# Autodesk Inventor assembly: Final Assembly
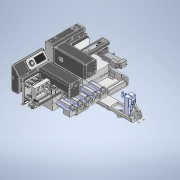
[picture p0: Inventor's stored thumbnail of the model, 180x180]
Saved by Autodesk Inventor 2022 (Build 260153000, 153)
## iProperties
Created: 2021-11-30
Part Number: Final Assembly
Document SubType Name: Assembly
Designer: efred
Author: efred
## Documents named in this file (59)
- C:\Users\efred\OneDrive - Imperial College London\Old Shit\ROBOICP\Final Assembly\Final Assembly.iam
- C:\Users\efred\OneDrive - Imperial College London\Old Shit\ROBOICP\Final Assembly\Linear Rail Base.ipt
- C:\Users\efred\OneDrive - Imperial College London\Old Shit\ROBOICP\Final Assembly\Linear Rail Carriage.ipt
- C:\Users\efred\OneDrive - Imperial College London\Old Shit\ROBOICP\Final Assembly\Linear Rail motor.ipt
- C:\Users\efred\OneDrive - Imperial College London\Old Shit\ROBOICP\Final Assembly\Linear Rail End Cap.ipt
- C:\Users\efred\OneDrive - Imperial College London\Old Shit\ROBOICP\Final Assembly\Linear Rail Front Plate.ipt
- C:\Users\efred\OneDrive - Imperial College London\Old Shit\ROBOICP\Final Assembly\endcap insert.ipt
- C:\Users\efred\OneDrive - Imperial College London\Old Shit\ROBOICP\Final Assembly\endcap insert_MIR.ipt
- C:\Users\efred\OneDrive - Imperial College London\Old Shit\ROBOICP\Final Assembly\backboard.ipt
- C:\Users\efred\OneDrive - Imperial College London\Old Shit\ROBOICP\Final Assembly\backboard_MIR.ipt
- C:\Users\efred\OneDrive - Imperial College London\Old Shit\ROBOICP\Final Assembly\Syringe adapter to rail.ipt
- C:\Users\efred\OneDrive - Imperial College London\Old Shit\ROBOICP\Final Assembly\SyringeHolder.ipt
- C:\Users\efred\OneDrive - Imperial College London\Old Shit\ROBOICP\Final Assembly\Guide rod bottom stand (independent).ipt
- C:\Users\efred\OneDrive - Imperial College London\Old Shit\ROBOICP\Final Assembly\Linear Rail Frame Bracket.ipt
- C:\Users\efred\OneDrive - Imperial College London\Old Shit\ROBOICP\Final Assembly\Linear Rail Frame Bracket_MIR.ipt
- C:\Users\efred\OneDrive - Imperial College London\Old Shit\ROBOICP\Final Assembly\Lower Support.ipt
- C:\Users\efred\OneDrive - Imperial College London\Old Shit\ROBOICP\Final Assembly\Lower Support_MIR.ipt
- C:\Users\efred\OneDrive - Imperial College London\Old Shit\ROBOICP\Final Assembly\Linear actuator piston.ipt
- C:\Users\efred\OneDrive - Imperial College London\Old Shit\ROBOICP\Final Assembly\linear actuator conrod.ipt
- C:\Users\efred\OneDrive - Imperial College London\Old Shit\ROBOICP\Final Assembly\6x250 steel rod.ipt
- C:\Users\efred\OneDrive - Imperial College London\Old Shit\ROBOICP\Final Assembly\cantilever.ipt
- C:\Users\efred\OneDrive - Imperial College London\Old Shit\ROBOICP\Final Assembly\Servo head assembly.iam
- C:\Users\efred\OneDrive - Imperial College London\Old Shit\ROBOICP\Final Assembly\Conrod.ipt
- C:\Users\efred\OneDrive - Imperial College London\Old Shit\ROBOICP\Final Assembly\Syringe Lower.ipt
- C:\Users\efred\OneDrive - Imperial College London\Old Shit\ROBOICP\Final Assembly\Plunger Assembly.iam
- C:\Users\efred\OneDrive - Imperial College London\Old Shit\ROBOICP\Final Assembly\Dilution Printer.iam
- C:\Users\efred\OneDrive - Imperial College London\Old Shit\ROBOICP\Final Assembly\Bed plate.ipt
- C:\Users\efred\OneDrive - Imperial College London\Old Shit\ROBOICP\Final Assembly\Nema17(SY42STH47-1684A)singelshaft.ipt
- C:\Users\efred\OneDrive - Imperial College London\Old Shit\ROBOICP\Final Assembly\Rotating Vial Holder EXP Slice.ipt
- C:\Users\efred\OneDrive - Imperial College London\Old Shit\ROBOICP\Final Assembly\small Vial.ipt
- C:\Users\efred\OneDrive - Imperial College London\Old Shit\ROBOICP\Final Assembly\L298N.ipt
- C:\Users\efred\OneDrive - Imperial College London\Old Shit\ROBOICP\Final Assembly\Reaction Printer.iam
- C:\Users\efred\OneDrive - Imperial College London\Old Shit\ROBOICP\Final Assembly\Raspberry Pi 3.ipt
- C:\Users\efred\OneDrive - Imperial College London\Old Shit\ROBOICP\Final Assembly\linear actuator.ipt
- C:\Users\efred\OneDrive - Imperial College London\Old Shit\ROBOICP\Final Assembly\Power brick assembly.iam
- C:\Users\efred\OneDrive - Imperial College London\Old Shit\ROBOICP\Final Assembly\printer power brick assembly.iam
- C:\Users\efred\OneDrive - Imperial College London\Old Shit\ROBOICP\Final Assembly\dilution system bracket.ipt
- C:\Users\efred\OneDrive - Imperial College London\Old Shit\ROBOICP\Final Assembly\dilution system bracket_MIR.ipt
- C:\Users\efred\OneDrive - Imperial College London\Old Shit\ROBOICP\Final Assembly\pivot module base.ipt
- C:\Users\efred\OneDrive - Imperial College London\Old Shit\ROBOICP\Final Assembly\pivot module stalk.ipt
- C:\Users\efred\OneDrive - Imperial College London\Old Shit\ROBOICP\Final Assembly\TB6600 - Driver Motor de Passo 4A.ipt
- C:\Users\efred\OneDrive - Imperial College London\Old Shit\ROBOICP\Final Assembly\persitaltic pump assembly.iam
- C:\Users\efred\OneDrive - Imperial College London\Old Shit\ROBOICP\Final Assembly\ArduinoMega_STEP_AP203.ipt
- C:\Users\efred\OneDrive - Imperial College London\Old Shit\ROBOICP\Final Assembly\electronics box.ipt
- C:\Users\efred\Downloads\Breadboard.ipt
- C:\Users\efred\OneDrive - Imperial College London\Old Shit\ROBOICP\Final Assembly\sump.ipt
- C:\Users\efred\Downloads\beaker holder.ipt
- C:\Users\efred\OneDrive - Imperial College London\Old Shit\ROBOICP\Final Assembly\Keyes KY 019 Montaj.ipt
- C:\Users\efred\OneDrive - Imperial College London\Old Shit\ROBOICP\Final Assembly\Micropippete mount assembly.iam
- C:\Users\efred\OneDrive - Imperial College London\Old Shit\ROBOICP\Final Assembly\Solids Feeder Head Assembly.iam
- C:\Users\efred\OneDrive - Imperial College London\Old Shit\ROBOICP\Final Assembly\male head_1.75R.ipt
- C:\Users\efred\OneDrive - Imperial College London\Old Shit\ROBOICP\Final Assembly\new top 4.0.ipt
- C:\Users\efred\OneDrive - Imperial College London\Old Shit\ROBOICP\Final Assembly\vial.ipt
- C:\Users\efred\OneDrive - Imperial College London\Old Shit\ROBOICP\Final Assembly\female mixing head.ipt
- C:\Users\efred\OneDrive - Imperial College London\Old Shit\ROBOICP\Final Assembly\Mixer.ipt
- C:\Users\efred\OneDrive - Imperial College London\Old Shit\ROBOICP\Final Assembly\vial holder 2.ipt
- C:\Users\efred\OneDrive - Imperial College London\Old Shit\ROBOICP\Final Assembly\hopper motor holder.ipt
- C:\Users\efred\OneDrive - Imperial College London\Old Shit\ROBOICP\Final Assembly\motor.ipt
- C:\Users\efred\OneDrive - Imperial College London\Old Shit\ROBOICP\Final Assembly\motor viber.ipt
## Components (80 placed, 58 different names)
1. Linear Rail Base:1 — Flush:1, Mate:1, Mate:2, Flush:2, Mate:3, Mate:4, Mate:5, Mate:6, Flush:6, Mate:18, Flush:13, Flush:70, Flush:71
2. Linear Rail Carriage:1 — Mate:5, Mate:6, Mate:14, Angle:2, Flush:9, Flush:10, Flush:12
3. Linear Rail motor:1 — Mate:7, Angle:1, Mate:8
4. Linear Rail End Cap:1 — Flush:2, Mate:3, Mate:4, Flush:3, Mate:126
5. Linear Rail Front Plate:1 — Flush:1, Mate:1, Mate:2, Mate:7, Angle:1, Mate:8, Mate:17, Mate:71, Mate:72, Flush:72, Mate:125
6. endcap insert:1 — Flush:4, Flush:5, Flush:15
7. endcap insert_MIR:1 — Mate:9, Mate:10, Mate:71, Mate:72, Flush:72, Mate:73, Mate:75
8. backboard:1 — Flush:7, Flush:71, Mate:73, Mate:74, Mate:79, Mate:80, Mate:81
9. backboard_MIR:1 — Mate:11, Flush:14, Flush:70, Mate:76, Mate:77, Mate:78, Mate:147, Flush:130
10. Syringe adapter to rail:1 — Mate:14, Angle:2, Flush:9, Flush:10, Mate:15, Mate:16, Mate:17, Mate:125, Mate:126
11. SyringeHolder:1 — Mate:15, Flush:12, Mate:16, Mate:45, Mate:46, Angle:3
12. Guide rod bottom stand (independent):1 — Mate:18, Flush:13, Mate:30, Mate:32, Mate:37, Mate:41, Mate:42, Mate:49, Flush:68, Mate:68, Mate:69, Mate:70, Mate:91, Flush:75, Mate:101, Flush:103, Mate:102, Flush:104
13. Linear Rail Frame Bracket:1 — Flush:15
14. Linear Rail Frame Bracket_MIR:1 — Mate:74, Mate:75
15. Lower Support:1 — Flush:16, Flush:17, Mate:79, Mate:80, Mate:81, Flush:81, Mate:160
16. Lower Support_MIR:1 — Flush:17, Flush:69, Mate:76, Mate:77, Mate:78, Angle:5, Mate:92, Flush:83, Flush:105, Mate:104, Mate:105, Mate:148, Flush:133, Flush:164
17. Linear actuator piston:1 — Mate:67, Mate:103
18. 6x250 steel rod:1 — Mate:30, Mate:43, Mate:70
19. cantilever:1 — Mate:32, Mate:39, Mate:66, Mate:69
20. Servo head assembly:1 [sub-assembly] — Mate:38, Mate:43, Mate:68, Mate:89, Mate:91
21. Conrod:1 — Mate:37, Mate:38, Mate:39
22. 6x250 steel rod:2 — Mate:41, Mate:42
23. Dilution Printer:1 [sub-assembly] — Flush:69, Mate:82, Mate:83, Mate:84, Angle:4, Angle:5, Mate:92, Flush:83, Flush:113, Mate:166, Mate:167, Mate:168
24. Bed plate:1 — Mate:55, Mate:56, Mate:57, Mate:82, Mate:83, Mate:84, Mate:86, Mate:144, Mate:145
25. Nema17(SY42STH47-1684A)singelshaft:1 — Mate:55, Mate:56, Mate:57, Mate:85
26. linear actuator conrod:1 — Flush:68, Mate:66, Mate:67
27. Rotating Vial Holder EXP Slice:1 — Mate:85, Mate:86, Angle:4, Mate:87, Mate:88
28. small Vial:1 — Mate:87, Mate:88, Mate:89
29. Reaction Printer:1 [sub-assembly] — Flush:81, Mate:159, Mate:160, Mate:171, Mate:172, Flush:177, Flush:178, Flush:180, Mate:173, Mate:174, Flush:181, Flush:182, Mate:177, Flush:184, Flush:188
30. Raspberry Pi 3:1 — Flush:158, Flush:159, Mate:158
31. linear actuator:1 — Mate:101, Flush:103, Mate:102, Flush:104, Mate:103
32. Power brick assembly:1 [sub-assembly] — Mate:106, Flush:106, Flush:107
33. dilution system bracket:1 — Flush:114, Flush:115, Flush:168, Mate:159
34. dilution system bracket_MIR:1 — Mate:123, Mate:124, Flush:167, Flush:173
35. pivot module base:1 — Flush:116, Flush:117
36. pivot module stalk:1 — Flush:118, Flush:119
37. small Vial:2 — Mate:144, Mate:145
38. persitaltic pump assembly:1 [sub-assembly] — Mate:147, Flush:130, Mate:148
39. ArduinoMega_STEP_AP203:1 — Mate:155, Mate:156, Mate:157
40. electronics box:1 — Mate:152, Flush:136, Flush:137, Mate:153, Mate:154, Mate:162, Tangent:5, Flush:156, Mate:161, Mate:156, Flush:159, Mate:158, Mate:163, Mate:164, Mate:165
41. Breadboard:2 — Mate:153, Flush:156, Mate:161, Flush:158, Mate:157
42. sump:1 — Flush:165, Flush:166, Flush:167, Flush:168
43. beaker holder:1 — Flush:174
44. Keyes KY 019 Montaj:1 — Mate:163, Mate:164, Mate:165
45. Micropippete mount assembly:1 [sub-assembly] — Mate:166, Mate:167, Mate:168
46. Solids Feeder Head Assembly:1 [sub-assembly] — Mate:171, Mate:172, Flush:177, Flush:179, Flush:180, Flush:189, Mate:188, Mate:189
47. male head_1.75R:1 — Mate:173, Mate:174, Flush:183, Mate:178
48. new top 4.0:1 — Flush:181, Flush:182, Mate:175, Mate:178, Flush:187, Mate:182, Mate:183, Flush:192, Mate:192
49. female mixing head:1 — Flush:187, Angle:6, Mate:190, Mate:191
50. Mixer:1 — Angle:6, Mate:190, Mate:191
51. vial holder 2:1 — Flush:188
52. hopper motor holder:1 — Flush:190, Flush:191, Mate:188, Mate:189, Mate:194, Flush:197
53. hopper motor holder:2 — Mate:182, Mate:183, Flush:192, Mate:185, Flush:194
54. motor:2 — Mate:185, Flush:194, Mate:186, Flush:195
55. motor viber:1 — Mate:186, Flush:195
56. motor:3 — Mate:194, Flush:197
57. motor viber:2
58. Syringe Lower:1 — Mate:45, Mate:46, Angle:3, Mate:47, Mate:48
59. Syringe Lower:2
60. Syringe Lower:3
61. Syringe Lower:4
62. Syringe Lower:5
63. Plunger Assembly:1 [sub-assembly] — Mate:47, Mate:48, Mate:49
64. Plunger Assembly:2 [sub-assembly]
65. Plunger Assembly:3 [sub-assembly]
66. Plunger Assembly:4 [sub-assembly]
67. Plunger Assembly:5 [sub-assembly]
68. printer power brick assembly:1 [sub-assembly] — Flush:105, Mate:104, Mate:105
69. printer power brick assembly:2 [sub-assembly] — Mate:106, Flush:106, Flush:107
70. L298N:1 — Mate:152, Flush:136, Flush:137
71. L298N:2
72. L298N:3 — Mate:155
73. TB6600 - Driver Motor de Passo 4A:1 — Mate:154, Mate:162, Tangent:5
74. TB6600 - Driver Motor de Passo 4A:2
75. vial:1 — Mate:175, Mate:177, Mate:192
76. vial:2
77. vial:3
78. vial:4
79. vial:5
80. vial:6
## Component patterns: (5 elements, first: Syringe Lower:1), (5 elements, first: Plunger Assembly:1), (2 elements, first: printer power brick assembly:1), (3 elements, first: L298N:1), (2 elements, first: TB6600 - Driver Motor de Passo 4A:1), (6 elements, first: vial:1)
## Relationships (181: Mate 107, Flush 67, Angle 6, Tangent 1)
- Flush:1: Linear Rail Base:1 ↔ Linear Rail Front Plate:1
- Mate:1 (3.2 mm): Linear Rail Base:1 ↔ Linear Rail Front Plate:1
- Mate:2: Linear Rail Base:1 ↔ Linear Rail Front Plate:1
- Flush:2: Linear Rail Base:1 ↔ Linear Rail End Cap:1
- Mate:3 (3.2 mm): Linear Rail Base:1 ↔ Linear Rail End Cap:1
- Mate:4: Linear Rail Base:1 ↔ Linear Rail End Cap:1
- Mate:5 (1 mm): Linear Rail Base:1 ↔ Linear Rail Carriage:1
- Mate:6: Linear Rail Base:1 ↔ Linear Rail Carriage:1
- Mate:7: Linear Rail motor:1 ↔ Linear Rail Front Plate:1
- Angle:1 (0 deg): Linear Rail motor:1 ↔ Linear Rail Front Plate:1
- Mate:8: Linear Rail motor:1 ↔ Linear Rail Front Plate:1
- Flush:3 (0.1 mm): Linear Rail End Cap:1
- Flush:4: endcap insert:1
- Flush:5: endcap insert:1
- Mate:9: endcap insert_MIR:1
- Mate:10: endcap insert_MIR:1
- Flush:6 (0.1 mm): Linear Rail Base:1
- Flush:7 (0.1 mm): backboard:1
- Mate:11 (0.1 mm): backboard_MIR:1
- Mate:14 (0.1 mm): Linear Rail Carriage:1 ↔ Syringe adapter to rail:1
- Angle:2 (0 deg): Linear Rail Carriage:1 ↔ Syringe adapter to rail:1
- Flush:9: Linear Rail Carriage:1 ↔ Syringe adapter to rail:1
- Flush:10: Linear Rail Carriage:1 ↔ Syringe adapter to rail:1
- Mate:15 (0.1 mm): Syringe adapter to rail:1 ↔ SyringeHolder:1
- Flush:12: Linear Rail Carriage:1 ↔ SyringeHolder:1
- Mate:16 (0.1 mm): Syringe adapter to rail:1 ↔ SyringeHolder:1
- Mate:17 (1 mm): Linear Rail Front Plate:1 ↔ Syringe adapter to rail:1
- Mate:18 (0.1 mm): Linear Rail Base:1 ↔ Guide rod bottom stand (independent):1
- Flush:13 (-252.9 mm): Linear Rail Base:1 ↔ Guide rod bottom stand (independent):1
- Flush:14 (0.1 mm): backboard_MIR:1
- Flush:15: endcap insert:1 ↔ Linear Rail Frame Bracket:1
- Flush:16: Lower Support:1
- Flush:17: Lower Support:1 ↔ Lower Support_MIR:1
- Mate:30 (0.1 mm): Guide rod bottom stand (independent):1 ↔ 6x250 steel rod:1
- Mate:32: Guide rod bottom stand (independent):1 ↔ cantilever:1
- Mate:37: Guide rod bottom stand (independent):1 ↔ Conrod:1
- Mate:38: Servo head assembly:1 ↔ Conrod:1
- Mate:39: cantilever:1 ↔ Conrod:1
- Mate:41 (0.1 mm): Guide rod bottom stand (independent):1 ↔ 6x250 steel rod:2
- Mate:42: Guide rod bottom stand (independent):1 ↔ 6x250 steel rod:2
- Mate:43: 6x250 steel rod:1 ↔ Servo head assembly:1
- Mate:45 (0.1 mm): SyringeHolder:1 ↔ Syringe Lower:1
- Mate:46: SyringeHolder:1 ↔ Syringe Lower:1
- Angle:3 (0 deg): SyringeHolder:1 ↔ Syringe Lower:1
- Mate:47: Syringe Lower:1 ↔ Plunger Assembly:1
- Mate:48 (9.6 mm): Syringe Lower:1 ↔ Plunger Assembly:1
- Mate:49: Guide rod bottom stand (independent):1 ↔ Plunger Assembly:1
- Mate:55 (0.1 mm): Bed plate:1 ↔ Nema17(SY42STH47-1684A)singelshaft:1
- Mate:56 (0.1 mm): Bed plate:1 ↔ Nema17(SY42STH47-1684A)singelshaft:1
- Mate:57 (0.1 mm): Bed plate:1 ↔ Nema17(SY42STH47-1684A)singelshaft:1
- Flush:68: Guide rod bottom stand (independent):1 ↔ linear actuator conrod:1
- Mate:66: cantilever:1 ↔ linear actuator conrod:1
- Mate:67: Linear actuator piston:1 ↔ linear actuator conrod:1
- Mate:68: Guide rod bottom stand (independent):1 ↔ Servo head assembly:1
- Mate:69: Guide rod bottom stand (independent):1 ↔ cantilever:1
- Mate:70: Guide rod bottom stand (independent):1 ↔ 6x250 steel rod:1
- Flush:69: Lower Support_MIR:1 ↔ Dilution Printer:1
- Flush:70: Linear Rail Base:1 ↔ backboard_MIR:1
- Flush:71: Linear Rail Base:1 ↔ backboard:1
- Mate:71 (0.1 mm): Linear Rail Front Plate:1 ↔ endcap insert_MIR:1
- Mate:72: Linear Rail Front Plate:1 ↔ endcap insert_MIR:1
- Flush:72: Linear Rail Front Plate:1 ↔ endcap insert_MIR:1
- Mate:73: endcap insert_MIR:1 ↔ backboard:1
- Mate:74: backboard:1 ↔ Linear Rail Frame Bracket_MIR:1
- Mate:75: endcap insert_MIR:1 ↔ Linear Rail Frame Bracket_MIR:1
- Mate:76 (0.1 mm): backboard_MIR:1 ↔ Lower Support_MIR:1
- Mate:77 (0.1 mm): backboard_MIR:1 ↔ Lower Support_MIR:1
- Mate:78 (0.1 mm): backboard_MIR:1 ↔ Lower Support_MIR:1
- Mate:79 (0.1 mm): backboard:1 ↔ Lower Support:1
- Mate:80 (0.1 mm): backboard:1 ↔ Lower Support:1
- Mate:81 (0.1 mm): backboard:1 ↔ Lower Support:1
- Mate:82 (0.1 mm): Dilution Printer:1 ↔ Bed plate:1
- Mate:83: Dilution Printer:1 ↔ Bed plate:1
- Mate:84: Dilution Printer:1 ↔ Bed plate:1
- Mate:85: Nema17(SY42STH47-1684A)singelshaft:1 ↔ Rotating Vial Holder EXP Slice:1
- Mate:86 (10 mm): Bed plate:1 ↔ Rotating Vial Holder EXP Slice:1
- Angle:4 (20 deg): Dilution Printer:1 ↔ Rotating Vial Holder EXP Slice:1
- Mate:87: Rotating Vial Holder EXP Slice:1 ↔ small Vial:1
- Mate:88 (0.1 mm): Rotating Vial Holder EXP Slice:1 ↔ small Vial:1
- Mate:89: Servo head assembly:1 ↔ small Vial:1
- Angle:5 (0 deg): Lower Support_MIR:1 ↔ Dilution Printer:1
- Mate:91: Guide rod bottom stand (independent):1 ↔ Servo head assembly:1
- Mate:92 (58 mm): Lower Support_MIR:1 ↔ Dilution Printer:1
- Flush:75 (0.1 mm): Guide rod bottom stand (independent):1
- Flush:81: Lower Support:1 ↔ Reaction Printer:1
- Flush:83 (108 mm): Lower Support_MIR:1 ↔ Dilution Printer:1
- Mate:101 (0.1 mm): Guide rod bottom stand (independent):1 ↔ linear actuator:1
- Flush:103: Guide rod bottom stand (independent):1 ↔ linear actuator:1
- Mate:102 (-50 mm): Guide rod bottom stand (independent):1 ↔ linear actuator:1
- Flush:104: Guide rod bottom stand (independent):1 ↔ linear actuator:1
- Mate:103: Linear actuator piston:1 ↔ linear actuator:1
- Flush:105: Lower Support_MIR:1 ↔ printer power brick assembly:1
- Mate:104 (0.1 mm): Lower Support_MIR:1 ↔ printer power brick assembly:1
- Mate:105 (0.1 mm): Lower Support_MIR:1 ↔ printer power brick assembly:1
- Mate:106 (1 mm): Power brick assembly:1 ↔ printer power brick assembly:2
- Flush:106: Power brick assembly:1 ↔ printer power brick assembly:2
- Flush:107: Power brick assembly:1 ↔ printer power brick assembly:2
- Flush:113 (0.1 mm): Dilution Printer:1
- Flush:114: dilution system bracket:1
- Flush:115: dilution system bracket:1
- Mate:123: dilution system bracket_MIR:1
- Mate:124: dilution system bracket_MIR:1
- Flush:116: pivot module base:1
- Flush:117 (0.1 mm): pivot module base:1
- Flush:118: pivot module stalk:1
- Flush:119: pivot module stalk:1
- Mate:125: Linear Rail Front Plate:1 ↔ Syringe adapter to rail:1
- Mate:126: Linear Rail End Cap:1 ↔ Syringe adapter to rail:1
- Mate:144: Bed plate:1 ↔ small Vial:2
- Mate:145 (0.1 mm): Bed plate:1 ↔ small Vial:2
- Mate:147 (0.1 mm): backboard_MIR:1 ↔ persitaltic pump assembly:1
- Flush:130 (15 mm): backboard_MIR:1 ↔ persitaltic pump assembly:1
- Mate:148 (0.1 mm): Lower Support_MIR:1 ↔ persitaltic pump assembly:1
- Flush:133 (0.1 mm): Lower Support_MIR:1
- Mate:152 (5 mm): electronics box:1 ↔ L298N:1
- Flush:136 (1 mm): electronics box:1 ↔ L298N:1
- Flush:137 (10 mm): electronics box:1 ↔ L298N:1
- Mate:153 (0.1 mm): electronics box:1 ↔ Breadboard:2
- Mate:154 (0.1 mm): electronics box:1 ↔ TB6600 - Driver Motor de Passo 4A:1
- Mate:162 (10 mm): electronics box:1 ↔ TB6600 - Driver Motor de Passo 4A:1
- Tangent:5: electronics box:1 ↔ TB6600 - Driver Motor de Passo 4A:1
- Flush:156 (1 mm): electronics box:1 ↔ Breadboard:2
- Mate:161 (1 mm): electronics box:1 ↔ Breadboard:2
- Mate:155 (5 mm): ArduinoMega_STEP_AP203:1 ↔ L298N:3
- Mate:156 (5 mm): ArduinoMega_STEP_AP203:1 ↔ electronics box:1
- Flush:158 (30 mm): Raspberry Pi 3:1 ↔ Breadboard:2
- Flush:159: Raspberry Pi 3:1 ↔ electronics box:1
- Mate:157 (1 mm): ArduinoMega_STEP_AP203:1 ↔ Breadboard:2
- Mate:158 (5 mm): Raspberry Pi 3:1 ↔ electronics box:1
- Flush:164 (0.1 mm): Lower Support_MIR:1
- Flush:165: sump:1
- Flush:166: sump:1
- Flush:167 (0.1 mm): dilution system bracket_MIR:1 ↔ sump:1
- Flush:168 (0.1 mm): dilution system bracket:1 ↔ sump:1
- Flush:173 (0.1 mm): dilution system bracket_MIR:1
- Flush:174: beaker holder:1
- Mate:159 (25 mm): Reaction Printer:1 ↔ dilution system bracket:1
- Mate:160 (30 mm): Lower Support:1 ↔ Reaction Printer:1
- Mate:163: electronics box:1 ↔ Keyes KY 019 Montaj:1
- Mate:164: electronics box:1 ↔ Keyes KY 019 Montaj:1
- Mate:165 (1 mm): electronics box:1 ↔ Keyes KY 019 Montaj:1
- Mate:166 (0.1 mm): Dilution Printer:1 ↔ Micropippete mount assembly:1
- Mate:167: Dilution Printer:1 ↔ Micropippete mount assembly:1
- Mate:168: Dilution Printer:1 ↔ Micropippete mount assembly:1
- Mate:171 (5 mm): Reaction Printer:1 ↔ Solids Feeder Head Assembly:1
- Mate:172 (0.1 mm): Reaction Printer:1 ↔ Solids Feeder Head Assembly:1
- Flush:177: Reaction Printer:1 ↔ Solids Feeder Head Assembly:1
- Flush:178 (0.1 mm): Reaction Printer:1
- Flush:179: Solids Feeder Head Assembly:1
- Flush:180 (0.1 mm): Reaction Printer:1 ↔ Solids Feeder Head Assembly:1
- Mate:173: Reaction Printer:1 ↔ male head_1.75R:1
- Mate:174 (0.1 mm): Reaction Printer:1 ↔ male head_1.75R:1
- Flush:181: Reaction Printer:1 ↔ new top 4.0:1
- Flush:182 (4 mm): Reaction Printer:1 ↔ new top 4.0:1
- Mate:175: new top 4.0:1 ↔ vial:1
- Mate:177 (0.1 mm): Reaction Printer:1 ↔ vial:1
- Flush:183: male head_1.75R:1
- Flush:184 (0.1 mm): Reaction Printer:1
- Mate:178 (1 mm): male head_1.75R:1 ↔ new top 4.0:1
- Flush:187: new top 4.0:1 ↔ female mixing head:1
- Flush:188: Reaction Printer:1 ↔ vial holder 2:1
- Flush:189 (0.1 mm): Solids Feeder Head Assembly:1
- Flush:190: hopper motor holder:1
- Flush:191: hopper motor holder:1
- Mate:182 (0.1 mm): new top 4.0:1 ↔ hopper motor holder:2
- Mate:183 (0.1 mm): new top 4.0:1 ↔ hopper motor holder:2
- Flush:192: new top 4.0:1 ↔ hopper motor holder:2
- Mate:185: hopper motor holder:2 ↔ motor:2
- Flush:194: hopper motor holder:2 ↔ motor:2
- Mate:186: motor:2 ↔ motor viber:1
- Flush:195: motor:2 ↔ motor viber:1
- Mate:188 (0.1 mm): Solids Feeder Head Assembly:1 ↔ hopper motor holder:1
- Mate:189: Solids Feeder Head Assembly:1 ↔ hopper motor holder:1
- Angle:6 (0 deg): female mixing head:1 ↔ Mixer:1
- Mate:190 (0.1 mm): female mixing head:1 ↔ Mixer:1
- Mate:191: female mixing head:1 ↔ Mixer:1
- Mate:192 (0.1 mm): new top 4.0:1 ↔ vial:1
- [Mate]: motor:3 ↔ motor viber:2
- [Flush]: motor:3 ↔ motor viber:2
- Mate:194: hopper motor holder:1 ↔ motor:3
- Flush:197: hopper motor holder:1 ↔ motor:3
## Named parameters: d456_d446 = 0 mm, d457_d447 = 0 mm
